# Autodesk Inventor assembly: Butterfly Drive Base
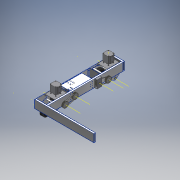
[picture p0: Inventor's stored thumbnail of the model, 180x180]
Saved by Autodesk Inventor 2019.4 (Build 234330000, 330)
## iProperties
Created: 2019-10-19
Part Number: Butterfly Drive Base
Document SubType Name: Assembly
Designer: Mark
Author: Mark
## Documents named in this file (27)
- C:\Users\admin\Desktop\FRC 2020 Engineering\GitHub\7738-CAD-prep\Butterfly drive\Butterfly Drive Base.iam
- C:\Users\admin\Desktop\FRC 2020 Engineering\GitHub\7738-CAD-prep\Butterfly drive\Butterfly Drive Module.iam
- C:\Users\admin\Desktop\FRC 2020 Engineering\GitHub\7738-CAD-prep\Butterfly drive\Side Extrusion.ipt
- C:\Users\admin\Desktop\FRC 2020 Engineering\GitHub\7738-CAD-prep\Butterfly drive\Module Plate 1.ipt
- C:\Users\admin\Desktop\FRC 2020 Engineering\GitHub\7738-CAD-prep\Butterfly drive\Back Extrusion 1.ipt
- C:\Users\admin\Desktop\FRC 2020 Engineering\GitHub\7738-CAD-prep\Butterfly drive\Bumper Plate.ipt
- C:\Users\admin\Desktop\FRC 2020 Engineering\GitHub\7738-CAD-prep\Butterfly drive\Side Front Extrusion.ipt
- C:\Users\admin\Desktop\FRC 2020 Engineering\GitHub\7738-CAD-prep\Butterfly drive\F6800Z 10mm ID Flange.ipt
- C:\Users\admin\Desktop\FRC 2020 Engineering\GitHub\7738-CAD-prep\2 Stage HD - CIM Sport.iam
- C:\Users\admin\Desktop\FRC 2020 Engineering\GitHub\7738-CAD-prep\am-0255 2.5inch CIM Motor.ipt
- C:\Users\admin\Desktop\FRC 2020 Engineering\GitHub\7738-CAD-prep\Butterfly drive\Spacer Extrusion.ipt
- C:\Users\admin\Desktop\FRC 2020 Engineering\GitHub\7738-CAD-prep\Butterfly drive\Butterfly Drive Base\Design Accelerator\Bevel Gears2.iam
- C:\Users\admin\Desktop\FRC 2020 Engineering\GitHub\7738-CAD-prep\Butterfly drive\Motor Protection Extrusion.ipt
- C:\Users\admin\Desktop\FRC 2020 Engineering\GitHub\7738-CAD-prep\Butterfly drive\Butterfly Drive Base\Design Accelerator\Synchronous Belts Transmission3.iam
- C:\Users\admin\Desktop\FRC 2020 Engineering\GitHub\7738-CAD-prep\transmition Axle Support.ipt
- C:\Users\admin\Desktop\FRC 2020 Engineering\GitHub\7738-CAD-prep\Butterfly drive\Pneumatic Connector.ipt
- C:\Users\admin\Desktop\FRC 2020 Engineering\GitHub\7738-CAD-prep\Butterfly drive\SDA 63 50 Full.iam
- C:\Users\admin\Desktop\FRC 2020 Engineering\GitHub\7738-CAD-prep\Butterfly drive\Front Motor Connector.ipt
- C:\Users\admin\Desktop\FRC 2020 Engineering\GitHub\7738-CAD-prep\Butterfly drive\Bevel holder.ipt
- C:\Users\admin\Desktop\FRC 2020 Engineering\GitHub\7738-CAD-prep\Butterfly drive\F10-18M Thrust Bearing.ipt
- C:\Users\admin\Desktop\FRC 2020 Engineering\GitHub\7738-CAD-prep\Butterfly drive\Motor Protection Extrusion_MIR.ipt
- C:\Users\admin\Desktop\FRC 2020 Engineering\GitHub\7738-CAD-prep\Butterfly drive\Spacer.ipt
- C:\Users\admin\Desktop\FRC 2020 Engineering\GitHub\7738-CAD-prep\Butterfly drive\F6004.ipt
- C:\Users\admin\Desktop\FRC 2020 Engineering\GitHub\7738-CAD-prep\Butterfly drive\F6802.ipt
- C:\Users\admin\Desktop\FRC 2020 Engineering\GitHub\7738-CAD-prep\Butterfly drive\Butterfly Drive Base\Design Accelerator\Shaft1.iam
- C:\Users\admin\Desktop\FRC 2020 Engineering\GitHub\7738-CAD-prep\Butterfly drive\Butterfly Drive Module_MIR1.iam
- C:\Users\admin\Desktop\FRC 2020 Engineering\GitHub\7738-CAD-prep\Butterfly drive\Butterfly Drive Base\Design Accelerator\Synchronous Belts Transmission4.iam
## Components (42 placed, 24 different names)
1. Butterfly Drive Module:1 [sub-assembly] — Mate:94, Mate:103, Angle:5, Mate:120
2. Side Extrusion:1 — Flush:7, Mate:10, Flush:8, Flush:9, Mate:20, Mate:26, Symmetry:1, Flush:10, Mate:29, Angle:2, Flush:11, Flush:15, Angle:3, Mate:47, Flush:18, Flush:19, Mate:63, Mate:69, Mate:70, Rotational:5, Rotational:6, Mate:91, Rotational:9, Mate:93, Mate:94, Angle:5, Mate:104, Mate:105, Angle:6, Mate:106, Flush:22, Mate:118, Flush:23
3. Back Extrusion 1:1 — Mate:118, Flush:23, Flush:24
4. Bumper Plate:1 — Mate:26, Mate:35, Mate:37, Flush:13, Mate:57, Rotational:7
5. Side Front Extrusion:1 — Flush:7, Mate:10, Flush:8, Symmetry:1, Mate:30, Mate:51, Mate:58, Flush:24
6. 2 Stage HD - CIM Sport:1 [sub-assembly] — Mate:15, Mate:16, Mate:17, Mate:20, Mate:33, Mate:34, Flush:15, Flush:16, Mate:51, Mate:54, Mate:55, Mate:56
7. am-0255 2.5inch CIM Motor:1 — Mate:15, Mate:16, Mate:17, Flush:17
8. 2 Stage HD - CIM Sport:2 [sub-assembly] — Mate:32, Flush:16, Mate:41, Flush:17, Mate:57
9. am-0255 2.5inch CIM Motor:2
10. Spacer Extrusion:2 — Flush:10, Mate:29, Mate:30, Mate:60, Symmetry:2
11. Bevel Gears:2 [sub-assembly] — Mate:33, Angle:2, Mate:34, Mate:43
12. Bevel Gears:3 [sub-assembly] — Mate:32, Mate:41, Mate:68, Mate:76, Mate:79, Mate:80, Mate:81
13. Spacer Extrusion:3 — Flush:11, Mate:35, Symmetry:2
14. Motor Protection Extrusion:2 — Mate:37, Flush:13, Mate:60, Mate:62, Mate:64, Mate:65, Flush:20, Flush:21
15. Synchronous Belts Transmission:1 [sub-assembly] — Mate:97, Mate:102, Angle:4
16. transmition Axle Support:1 — Mate:47, Flush:18, Mate:70, Rotational:3, Mate:97, Angle:4
17. Pneumatic Connector:1 — Mate:58, Flush:19, Rigid:1, Mate:69, Mate:82, Mate:83, Mate:84, Mate:85, Mate:86, Mate:87, Mate:88, Mate:89
18. SDA 63 50 Full:1 [sub-assembly] — Rigid:1, Mate:98, Mate:99
19. Front Motor Connector:1 — Mate:62, Mate:63, Mate:64, Mate:90
20. Bevel holder:1 — Mate:65, Mate:76, Mate:78, Flush:20, Rotational:1, Rotational:2
21. F10-18M Thrust Bearing:1 — Mate:80, Mate:81
22. Motor Protection Extrusion_MIR:1 — Flush:21, Mate:90, Mate:91
23. F6800Z 10mm ID Flange:3 — Rotational:1
24. F6800Z 10mm ID Flange:4 — Rotational:2
25. F6800Z 10mm ID Flange:5 — Rotational:3
26. F6800Z 10mm ID Flange:7 — Rotational:5
27. Spacer:1 — Mate:82, Mate:83
28. Spacer:2 — Mate:84, Mate:85
29. Spacer:3 — Mate:88, Mate:89
30. Spacer:4 — Mate:86, Mate:87
31. F6004:1 — Rotational:6
32. F6802:1 — Rotational:7, Rotational:8
33. Shaft:1 [sub-assembly] — Rotational:8, Mate:92, Mate:102, Mate:103
34. F6004:2 — Rotational:9
35. Butterfly Drive Module_MIR1:1 [sub-assembly] — Mate:104, Mate:105, Angle:6, Mate:119
36. Pneumatic Connector:2 — Mate:106, Flush:22, Mate:115, Mate:116, Mate:117
37. SDA 63 50 Full:2 [sub-assembly] — Mate:107, Mate:108, Mate:109, Mate:110, Mate:111, Mate:112, Mate:113, Mate:114
38. Spacer:5 — Mate:109, Mate:112, Mate:115, Mate:116
39. Spacer:6 — Mate:108, Mate:114, Mate:117
40. Spacer:7 — Mate:107, Mate:111
41. Spacer:8 — Mate:110, Mate:113
42. Synchronous Belts Transmission:2 [sub-assembly]
## Relationships (107: Mate 75, Flush 16, RevoluteJoint 8, Angle 5, Symmetry 2, WeldJoint 1)
- Flush:7: Side Extrusion:1 ↔ Side Front Extrusion:1
- Mate:10: Side Extrusion:1 ↔ Side Front Extrusion:1
- Flush:8: Side Extrusion:1 ↔ Side Front Extrusion:1
- Flush:9 (-18.548 mm): Side Extrusion:1
- Mate:15: 2 Stage HD - CIM Sport:1 ↔ am-0255 2.5inch CIM Motor:1
- Mate:16: 2 Stage HD - CIM Sport:1 ↔ am-0255 2.5inch CIM Motor:1
- Mate:17 (0.6 mm): 2 Stage HD - CIM Sport:1 ↔ am-0255 2.5inch CIM Motor:1
- Mate:20 (0.6 mm): Side Extrusion:1 ↔ 2 Stage HD - CIM Sport:1
- [Mate]: 2 Stage HD - CIM Sport:2 ↔ am-0255 2.5inch CIM Motor:2
- [Mate]: 2 Stage HD - CIM Sport:2 ↔ am-0255 2.5inch CIM Motor:2
- [Mate] (0.6 mm): 2 Stage HD - CIM Sport:2 ↔ am-0255 2.5inch CIM Motor:2
- Mate:26 (125 mm): Side Extrusion:1 ↔ Bumper Plate:1
- Symmetry:1: Side Extrusion:1 ↔ Side Front Extrusion:1
- Flush:10: Side Extrusion:1 ↔ Spacer Extrusion:2
- Mate:29: Side Extrusion:1 ↔ Spacer Extrusion:2
- Mate:30 (270 mm): Side Front Extrusion:1 ↔ Spacer Extrusion:2
- Mate:32: 2 Stage HD - CIM Sport:2 ↔ Bevel Gears:3
- Mate:33: 2 Stage HD - CIM Sport:1 ↔ Bevel Gears:2
- Angle:2 (180 deg): Side Extrusion:1 ↔ Bevel Gears:2
- Mate:34 (2 mm): 2 Stage HD - CIM Sport:1 ↔ Bevel Gears:2
- Flush:11: Side Extrusion:1 ↔ Spacer Extrusion:3
- Mate:35: Bumper Plate:1 ↔ Spacer Extrusion:3
- Mate:37: Bumper Plate:1 ↔ Motor Protection Extrusion:2
- Flush:13 (3 mm): Bumper Plate:1 ↔ Motor Protection Extrusion:2
- Flush:15 (26.1875 mm): Side Extrusion:1 ↔ 2 Stage HD - CIM Sport:1
- Flush:16: 2 Stage HD - CIM Sport:1 ↔ 2 Stage HD - CIM Sport:2
- Mate:41 (2 mm): 2 Stage HD - CIM Sport:2 ↔ Bevel Gears:3
- Mate:43: Bevel Gears:2
- Angle:3 (0 deg): Side Extrusion:1
- Flush:17: am-0255 2.5inch CIM Motor:1 ↔ 2 Stage HD - CIM Sport:2
- Mate:47: Side Extrusion:1 ↔ transmition Axle Support:1
- Flush:18: Side Extrusion:1 ↔ transmition Axle Support:1
- Mate:51 (374.508 mm): Side Front Extrusion:1 ↔ 2 Stage HD - CIM Sport:1
- Mate:54: 2 Stage HD - CIM Sport:1
- Mate:55: 2 Stage HD - CIM Sport:1
- Mate:56: 2 Stage HD - CIM Sport:1
- Mate:57 (13.375 mm): Bumper Plate:1 ↔ 2 Stage HD - CIM Sport:2
- Mate:58 (25 mm): Side Front Extrusion:1 ↔ Pneumatic Connector:1
- Flush:19 (-3 mm): Side Extrusion:1 ↔ Pneumatic Connector:1
- Rigid:1 [WeldJoint] (-20 mm): Pneumatic Connector:1 ↔ SDA 63 50 Full:1
- Mate:60 (100 mm): Spacer Extrusion:2 ↔ Motor Protection Extrusion:2
- Mate:62: Motor Protection Extrusion:2 ↔ Front Motor Connector:1
- Mate:63 (61 mm): Side Extrusion:1 ↔ Front Motor Connector:1
- Mate:64 (70 mm): Motor Protection Extrusion:2 ↔ Front Motor Connector:1
- Mate:65: Motor Protection Extrusion:2 ↔ Bevel holder:1
- Mate:68: Bevel Gears:3
- Mate:69: Side Extrusion:1 ↔ Pneumatic Connector:1
- Mate:70 (295.226 mm): Side Extrusion:1 ↔ transmition Axle Support:1
- Mate:76 (6.9 mm): Bevel Gears:3 ↔ Bevel holder:1
- Mate:78: Bevel holder:1
- Mate:79: Bevel Gears:3
- Flush:20 (-0.924 mm): Motor Protection Extrusion:2 ↔ Bevel holder:1
- Mate:80 (0.2 mm): Bevel Gears:3 ↔ F10-18M Thrust Bearing:1
- Mate:81: Bevel Gears:3 ↔ F10-18M Thrust Bearing:1
- Rotational:1 [RevoluteJoint]: Bevel holder:1 ↔ F6800Z 10mm ID Flange:3
- Rotational:2 [RevoluteJoint]: Bevel holder:1 ↔ F6800Z 10mm ID Flange:4
- Rotational:3 [RevoluteJoint]: transmition Axle Support:1 ↔ F6800Z 10mm ID Flange:5
- Rotational:5 [RevoluteJoint]: Side Extrusion:1 ↔ F6800Z 10mm ID Flange:7
- Mate:82: Pneumatic Connector:1 ↔ Spacer:1
- Mate:83: Pneumatic Connector:1 ↔ Spacer:1
- Mate:84: Pneumatic Connector:1 ↔ Spacer:2
- Mate:85: Pneumatic Connector:1 ↔ Spacer:2
- Mate:86: Pneumatic Connector:1 ↔ Spacer:4
- Mate:87: Pneumatic Connector:1 ↔ Spacer:4
- Mate:88: Pneumatic Connector:1 ↔ Spacer:3
- Mate:89: Pneumatic Connector:1 ↔ Spacer:3
- Rotational:6 [RevoluteJoint]: Side Extrusion:1 ↔ F6004:1
- Flush:21: Motor Protection Extrusion:2 ↔ Motor Protection Extrusion_MIR:1
- Mate:90: Front Motor Connector:1 ↔ Motor Protection Extrusion_MIR:1
- Mate:91: Side Extrusion:1 ↔ Motor Protection Extrusion_MIR:1
- Rotational:7 [RevoluteJoint]: Bumper Plate:1 ↔ F6802:1
- Rotational:8 [RevoluteJoint]: F6802:1 ↔ Shaft:1
- Rotational:9 [RevoluteJoint]: Side Extrusion:1 ↔ F6004:2
- Mate:92: Shaft:1
- Mate:93: Side Extrusion:1
- Mate:97 (3 mm): Synchronous Belts Transmission:1 ↔ transmition Axle Support:1
- Mate:94 (6 mm): Butterfly Drive Module:1 ↔ Side Extrusion:1
- Mate:98: SDA 63 50 Full:1
- Mate:99: SDA 63 50 Full:1
- Mate:100
- Mate:101
- Mate:102: Synchronous Belts Transmission:1 ↔ Shaft:1
- Angle:4 (-13.98 deg): Synchronous Belts Transmission:1 ↔ transmition Axle Support:1
- Mate:103: Butterfly Drive Module:1 ↔ Shaft:1
- Angle:5 (30 deg): Butterfly Drive Module:1 ↔ Side Extrusion:1
- Symmetry:2: Spacer Extrusion:2 ↔ Spacer Extrusion:3
- Mate:104: Side Extrusion:1 ↔ Butterfly Drive Module_MIR1:1
- Mate:105 (6 mm): Side Extrusion:1 ↔ Butterfly Drive Module_MIR1:1
- Angle:6 (-30 deg): Side Extrusion:1 ↔ Butterfly Drive Module_MIR1:1
- Mate:106: Side Extrusion:1 ↔ Pneumatic Connector:2
- Flush:22: Side Extrusion:1 ↔ Pneumatic Connector:2
- Mate:107: SDA 63 50 Full:2 ↔ Spacer:7
- Mate:108: SDA 63 50 Full:2 ↔ Spacer:6
- Mate:109: SDA 63 50 Full:2 ↔ Spacer:5
- Mate:110: SDA 63 50 Full:2 ↔ Spacer:8
- Mate:111: SDA 63 50 Full:2 ↔ Spacer:7
- Mate:112: SDA 63 50 Full:2 ↔ Spacer:5
- Mate:113: SDA 63 50 Full:2 ↔ Spacer:8
- Mate:114: SDA 63 50 Full:2 ↔ Spacer:6
- Mate:115: Pneumatic Connector:2 ↔ Spacer:5
- Mate:116: Pneumatic Connector:2 ↔ Spacer:5
- Mate:117: Pneumatic Connector:2 ↔ Spacer:6
- Mate:118: Side Extrusion:1 ↔ Back Extrusion 1:1
- Flush:23: Side Extrusion:1 ↔ Back Extrusion 1:1
- Flush:24: Back Extrusion 1:1 ↔ Side Front Extrusion:1
- Mate:119: Butterfly Drive Module_MIR1:1
- Mate:120: Butterfly Drive Module:1
## Named parameters: Height = 70 mm, ExtSta = 1 deg, ModuleAngle = 10 deg, d58_d50 = 0.6 mm, d59_d48 = 0 mm, d60_d49 = 0 mm
